# Autodesk Inventor assembly: ArmRotator
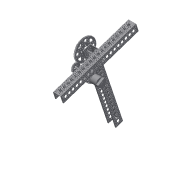
[picture p0: Inventor's stored thumbnail of the model, 180x180]
Saved by Autodesk Inventor 2018 (Build 220112000, 112)
## iProperties
Created: 2017-12-21
Part Number: ArmRotator
Document SubType Name: Assembly
Designer: ball
Author: ball
## Documents named in this file (8)
- C:\FTC\FTC8863CAD\2017Robot\ArmRotator.iam
- C:\FTC\FTC8863CAD\Actobotics\585 parts\585458.ipt
- C:\FTC\FTC8863CAD\Actobotics\634 parts\634082.ipt
- C:\FTC\FTC8863CAD\Andymark\am-2964NeveRest+40.ipt
- C:\FTC\FTC8863CAD\Actobotics\555 parts\555116.ipt
- C:\FTC\FTC8863CAD\Actobotics\545 parts\545360.ipt
- C:\FTC\FTC8863CAD\Actobotics\615 parts\615238.ipt
- C:\FTC\FTC8863CAD\Actobotics\615 parts\615190.ipt
## Components (9 placed, 7 different names)
1. 585458:2 — Mate:1, Mate:2, Mate:3, Angle:1
2. 585458:3 — Mate:1, Mate:2, Flush:1, Mate:13, Mate:16, Mate:17, Angle:1
3. 634082:1 — Mate:3, Flush:1, Mate:14, Flush:3
4. am-2964NeveRest+40:1 — Mate:10, Flush:2, Mate:15, Flush:4
5. 555116:1 — Mate:4, Mate:5, Mate:6, Flush:2
6. 555116:2 — Mate:7, Mate:8, Mate:9, Mate:10
7. 545360:1 — Mate:4, Mate:5, Mate:6, Mate:7, Mate:8, Mate:9, Mate:13, Mate:16, Mate:17
8. 615238:1 — Mate:14, Flush:3
9. 615190:1 — Mate:15, Flush:4
## Relationships (20: Mate 15, Flush 4, Angle 1)
- Mate:1: 585458:2 ↔ 585458:3
- Mate:2: 585458:2 ↔ 585458:3
- Mate:3: 585458:2 ↔ 634082:1
- Flush:1: 585458:3 ↔ 634082:1
- Mate:4: 555116:1 ↔ 545360:1
- Mate:5: 555116:1 ↔ 545360:1
- Mate:6: 555116:1 ↔ 545360:1
- Mate:7: 555116:2 ↔ 545360:1
- Mate:8: 555116:2 ↔ 545360:1
- Mate:9: 555116:2 ↔ 545360:1
- Mate:10: am-2964NeveRest+40:1 ↔ 555116:2
- Flush:2 (38.1 mm): am-2964NeveRest+40:1 ↔ 555116:1
- Mate:13: 585458:3 ↔ 545360:1
- Mate:14: 634082:1 ↔ 615238:1
- Flush:3 (38.1 mm): 634082:1 ↔ 615238:1
- Mate:15: am-2964NeveRest+40:1 ↔ 615190:1
- Flush:4 (7.62 mm): am-2964NeveRest+40:1 ↔ 615190:1
- Mate:16: 585458:3 ↔ 545360:1
- Mate:17: 585458:3 ↔ 545360:1
- Angle:1 (90 deg): 585458:2 ↔ 585458:3
